# Autodesk Inventor assembly: Assembly1
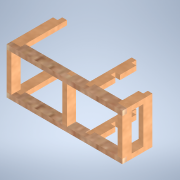
[picture p0: Inventor's stored thumbnail of the model, 180x180]
Saved by Autodesk Inventor 2022 (Build 260153000, 153)
## iProperties
Created: 2021-12-11
Part Number: Assembly1
Document SubType Name: Assembly
Designer: dangl
Author: dangl
## Documents named in this file (5)
- C:\Users\dangl\Documents\WoodWork\WorkBench\Assembly1.iam
- C:\Users\dangl\Documents\Ender3 Pro\My Prints\SmartVentCover\beam1.ipt
- C:\Users\dangl\Documents\WoodWork\WorkBench\beam2.ipt
- C:\Users\dangl\Documents\WoodWork\WorkBench\beam3.ipt
- C:\Users\dangl\Documents\WoodWork\WorkBench\beam4.ipt
## Components (12 placed, 4 different names)
1. beam1:1 — Mate:4, Mate:5, Mate:6, Flush:1, Flush:9, Mate:11, Mate:12, Flush:12, Mate:13
2. beam1:2 — Mate:1, Mate:2, Mate:3, Flush:2, Flush:3, Flush:4, Flush:5, Flush:6, Flush:8, Mate:8, Flush:11, Mate:9, Mate:10, Flush:15
3. beam2:1 — Mate:1, Mate:2, Mate:3, Mate:4, Mate:5, Mate:6
4. beam2:2 — Flush:1, Flush:2, Flush:3, Flush:13, Flush:14, Mate:14
5. beam2:3 — Flush:4, Flush:5, Flush:6, Flush:7, Mate:7, Flush:10
6. beam2:4 — Flush:9, Mate:7, Flush:10
7. beam2:5 — Flush:7, Flush:8, Mate:8
8. beam3:1 — Flush:11, Mate:9, Mate:10
9. beam3:2 — Mate:11, Mate:12
10. beam4:1 — Flush:12, Mate:13, Flush:13, Flush:16, Mate:15, Flush:17
11. beam4:2 — Flush:14, Flush:15, Mate:14
12. beam2:6 — Flush:16, Mate:15, Flush:17
## Relationships (32: Flush 17, Mate 15)
- Mate:1: beam1:2 ↔ beam2:1
- Mate:2: beam1:2 ↔ beam2:1
- Mate:3: beam1:2 ↔ beam2:1
- Mate:4: beam1:1 ↔ beam2:1
- Mate:5: beam1:1 ↔ beam2:1
- Mate:6: beam1:1 ↔ beam2:1
- Flush:1: beam1:1 ↔ beam2:2
- Flush:2: beam1:2 ↔ beam2:2
- Flush:3: beam1:2 ↔ beam2:2
- Flush:4: beam1:2 ↔ beam2:3
- Flush:5: beam1:2 ↔ beam2:3
- Flush:6: beam1:2 ↔ beam2:3
- Flush:7: beam2:3 ↔ beam2:5
- Flush:8: beam1:2 ↔ beam2:5
- Flush:9: beam1:1 ↔ beam2:4
- Mate:7: beam2:3 ↔ beam2:4
- Flush:10: beam2:3 ↔ beam2:4
- Mate:8: beam1:2 ↔ beam2:5
- Flush:11: beam1:2 ↔ beam3:1
- Mate:9: beam1:2 ↔ beam3:1
- Mate:10: beam1:2 ↔ beam3:1
- Mate:11: beam1:1 ↔ beam3:2
- Mate:12: beam1:1 ↔ beam3:2
- Flush:12: beam1:1 ↔ beam4:1
- Mate:13: beam1:1 ↔ beam4:1
- Flush:13: beam2:2 ↔ beam4:1
- Flush:14: beam2:2 ↔ beam4:2
- Flush:15: beam1:2 ↔ beam4:2
- Mate:14: beam2:2 ↔ beam4:2
- Flush:16: beam4:1 ↔ beam2:6
- Mate:15: beam4:1 ↔ beam2:6
- Flush:17: beam4:1 ↔ beam2:6
